# Autodesk Inventor assembly: Test_Rig_Assembly
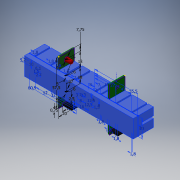
[picture p0: Inventor's stored thumbnail of the model, 180x180]
Saved by Autodesk Inventor 2016 (Build 200138000, 138)
## iProperties
Created: 2015-05-19
Part Number: Test_Rig_Assembly
Document SubType Name: Assembly
Designer: Openlab
Author: Openlab
## Documents named in this file (4)
- D:\Alexey\HS-Spectrophotometer\parts\Test\Assembly.iam
- D:\Alexey\HS-Spectrophotometer\parts\Test\Distance_test_rig.ipt
- D:\Alexey\HS-Spectrophotometer\parts\Test\LED_board.ipt
- D:\Alexey\HS-Spectrophotometer\parts\Test\Sensor_board.ipt
## Components (3 placed, 3 different names)
1. Distance_test_rig:1 — Mate:1, Mate:2, Mate:3, Mate:4
2. LED_board:1 — Mate:1, Mate:2
3. Sensor_board:1 — Mate:3, Mate:4
## Relationships (4: Mate 4)
- Mate:1: Distance_test_rig:1 ↔ LED_board:1
- Mate:2: Distance_test_rig:1 ↔ LED_board:1
- Mate:3: Distance_test_rig:1 ↔ Sensor_board:1
- Mate:4: Distance_test_rig:1 ↔ Sensor_board:1
